# Autodesk Inventor assembly: brake_light_top
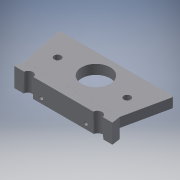
[picture p0: Inventor's stored thumbnail of the model, 180x180]
Saved by Autodesk Inventor 2019 (Build 230136000, 136)
## iProperties
Created: 2019-09-06
Part Number: brake_light_top
Document SubType Name: Assembly
Designer: steve
Author: steve
## Documents named in this file (3)
- C:\Users\steve\Documents\GitHub\Motorcycle\CAD Files\brake_light_top.iam
- C:\Users\steve\Documents\GitHub\Motorcycle\CAD Files\Bar_Mount_Bottom.ipt
- C:\Users\steve\Documents\GitHub\Motorcycle\CAD Files\brake_Light_top_mount.ipt
## Components (2 placed, 2 different names)
1. Bar_Mount_Bottom:1 — Rigid:1
2. Brake_Light_Base_Plate:1 — Rigid:1
## Relationships (1: WeldJoint 1)
- Rigid:1 [WeldJoint]: Bar_Mount_Bottom:1 ↔ Brake_Light_Base_Plate:1
